# Autodesk Inventor assembly: Side Bumper
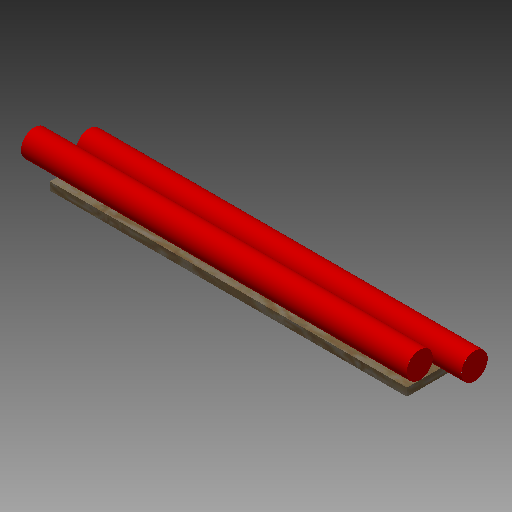
[picture p0: Inventor's stored thumbnail of the model, 512x512]
Saved by Autodesk Inventor 2018 (Build 220112000, 112)
## iProperties
Created: 2018-01-17
Part Number: Side Bumper
Document SubType Name: Assembly
Designer: Apple
Author: Apple
## Documents named in this file (3)
- C:\Users\Apple\Documents\Inventor\2018 PowerUp\Bumper\Side Bumper.iam
- C:\Users\Apple\Documents\Inventor\2018 PowerUp\Bumper\Side Board.ipt
- C:\Users\Apple\Documents\Inventor\2018 PowerUp\Bumper\Noodle.ipt
## Components (3 placed, 2 different names)
1. Side Board:1 — Flush:1, Flush:2, Tangent:1, Tangent:3, Mate:1
2. Noodle:1 — Flush:1, Tangent:2, Tangent:3
3. Noodle:2 — Flush:2, Tangent:1, Tangent:2, Mate:1
## Relationships (6: Tangent 3, Flush 2, Mate 1)
- Flush:1: Side Board:1 ↔ Noodle:1
- Flush:2: Side Board:1 ↔ Noodle:2
- Tangent:1: Side Board:1 ↔ Noodle:2
- Tangent:2: Noodle:1 ↔ Noodle:2
- Tangent:3: Side Board:1 ↔ Noodle:1
- Mate:1 (-32.814 mm): Side Board:1 ↔ Noodle:2
